# Autodesk Inventor assembly: u106_long_design_newbearing
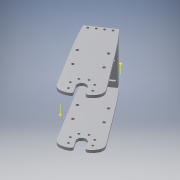
[picture p0: Inventor's stored thumbnail of the model, 180x180]
Saved by Autodesk Inventor 2018 (Build 220112000, 112)
## iProperties
Created: 2017-02-17
Part Number: u106_long_design_newbearing
Document SubType Name: Assembly
Designer: steve
Author: steve
## Documents named in this file (3)
- C:\Users\etd\Dropbox\SigmaBan\SigmaBanV2.1\Ulong\u106_long_design_newbearing.iam
- C:\Users\etd\Dropbox\SigmaBan\SigmaBanV2.1\Ulong\new_side_u106_long_design.ipt
- C:\Users\etd\Dropbox\SigmaBan\SigmaBanV2.1\Ulong\new_base_u106_long_newbearing.ipt
## Components (3 placed, 2 different names)
1. new_base_u106_long_newbearing:1 — Mate:2, Mate:3, Mate:4, Mate:5, Mate:6, Mate:7
2. new_side_u106_long_design:1 — Mate:2, Mate:3, Mate:4
3. new_side_u106_long_design:2 — Mate:5, Mate:6, Mate:7
## Relationships (6: Mate 6)
- Mate:2: new_base_u106_long_newbearing:1 ↔ new_side_u106_long_design:1
- Mate:3: new_base_u106_long_newbearing:1 ↔ new_side_u106_long_design:1
- Mate:4: new_base_u106_long_newbearing:1 ↔ new_side_u106_long_design:1
- Mate:5: new_base_u106_long_newbearing:1 ↔ new_side_u106_long_design:2
- Mate:6: new_base_u106_long_newbearing:1 ↔ new_side_u106_long_design:2
- Mate:7: new_base_u106_long_newbearing:1 ↔ new_side_u106_long_design:2
